# Autodesk Inventor assembly: engranaje worm
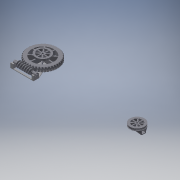
[picture p0: Inventor's stored thumbnail of the model, 180x180]
Saved by Autodesk Inventor 2016 (Build 200138000, 138)
## iProperties
Created: 2016-07-30
Part Number: engranaje worm
Document SubType Name: Assembly
Designer: Admin
Author: Admin
## Documents named in this file (6)
- C:\Users\Admin\Documents\diseños autodesk dimer\engranaje worm.iam
- C:\Users\Admin\Documents\diseños autodesk dimer\soporte worm.ipt
- C:\Users\Admin\Documents\diseños autodesk dimer\worm gear\Design Accelerator\Worm Gears2.iam
- C:\Users\Admin\Documents\diseños autodesk dimer\worm gear\Design Accelerator\Worm Gear2.ipt
- C:\Users\Admin\Documents\diseños autodesk dimer\worm gear\Design Accelerator\Spur Gears2.iam
- C:\Users\Admin\Documents\diseños autodesk dimer\worm gear\Design Accelerator\Spur Gears1.iam
## Components (5 placed, 4 different names)
1. soporte worm:1 — Mate:4, Mate:5
2. Worm Gears:1 [sub-assembly]
3. Worm Gear:1 — Mate:1, Mate:2, Flush:1, Mate:4, Mate:5
4. Spur Gears:1 [sub-assembly] — Flush:2, Mate:3
5. Spur Gears:2 [sub-assembly] — Mate:1, Mate:2, Flush:1, Flush:2, Mate:3
## Relationships (7: Mate 5, Flush 2)
- Mate:1: Worm Gear:1 ↔ Spur Gears:2
- Mate:2: Worm Gear:1 ↔ Spur Gears:2
- Flush:1: Worm Gear:1 ↔ Spur Gears:2
- Flush:2: Spur Gears:1 ↔ Spur Gears:2
- Mate:3 (400 mm): Spur Gears:1 ↔ Spur Gears:2
- Mate:4: soporte worm:1 ↔ Worm Gear:1
- Mate:5 (8 mm): soporte worm:1 ↔ Worm Gear:1
